# Autodesk Inventor assembly: Assembly4
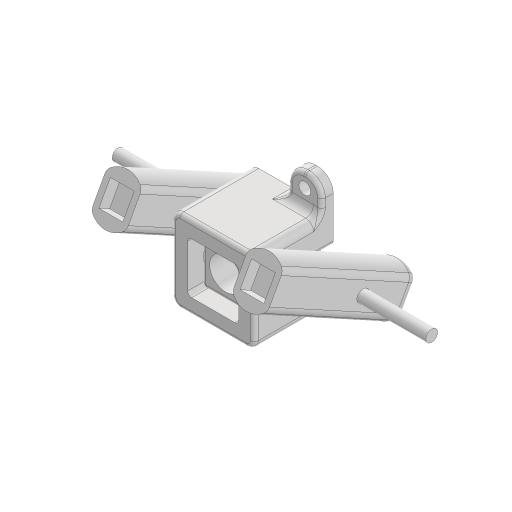
[picture p0: Inventor's stored thumbnail of the model, 512x512]
Saved by Autodesk Inventor 2024 (Build 280153000, 153)
## iProperties
Created: 2023-11-07
Part Number: Assembly4
Document SubType Name: Assembly
Designer: bonju
Author: bonju
## Documents named in this file (5)
- C:\Users\moonshot\Desktop\ikisawa\ikisawa\experiment8_standing\leg_unit\leg_unit.iam
- C:\Users\moonshot\Desktop\ikisawa\ikisawa\experiment8_standing\leg_unit\parent_ver.1.ipt
- C:\Users\moonshot\Desktop\ikisawa\ikisawa\experiment8_standing\leg_unit\cover.ver1.ipt
- C:\Users\moonshot\Desktop\ikisawa\ikisawa\experiment8_standing\leg_unit\shaft_leg.ipt
- C:\Users\moonshot\Desktop\ikisawa\ikisawa\experiment8_standing\leg_unit\leg.ipt
## Components (5 placed, 4 different names)
1. parent_ver.1:1 — スライダ:1, メイト:11, メイト:12
2. cover.ver1:1 — メイト:1, メイト:2, フラッシュ:1, メイト:9, メイト:10, スライダ:1
3. shaft_leg:1 — メイト:3, メイト:4, メイト:11, メイト:12
4. leg:1 — メイト:3, メイト:10
5. leg:2 — メイト:4, メイト:9
## Relationships (10: Mate 8, Flush 1, TranslationJoint 1)
- メイト:1 [Mate]: cover.ver1:1
- メイト:2 [Mate]: cover.ver1:1
- フラッシュ:1 [Flush]: cover.ver1:1
- メイト:3 [Mate]: shaft_leg:1 ↔ leg:1
- メイト:4 [Mate]: shaft_leg:1 ↔ leg:2
- メイト:9 [Mate] (3 mm): cover.ver1:1 ↔ leg:2
- メイト:10 [Mate] (3 mm): cover.ver1:1 ↔ leg:1
- スライダ:1 [TranslationJoint] (1.5 mm): parent_ver.1:1 ↔ cover.ver1:1
- メイト:11 [Mate]: parent_ver.1:1 ↔ shaft_leg:1
- メイト:12 [Mate]: parent_ver.1:1 ↔ shaft_leg:1
